# Autodesk Inventor assembly: Assem3omni
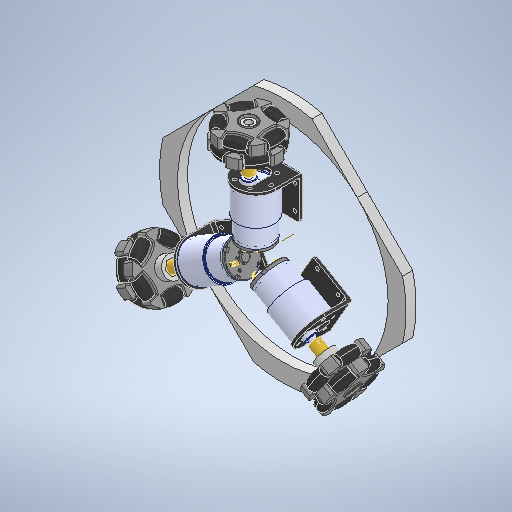
[picture p0: Inventor's stored thumbnail of the model, 512x512]
Saved by Autodesk Inventor 2025.1 (Build 291241000, 241)
## iProperties
Created: 2025-05-09
Part Number: Assem3omni
Document SubType Name: Assembly
Designer: User
Author: User
## Documents named in this file (3)
- D:\One Drive\OneDrive - Politeknik Sultan Salahuddin Abdul Aziz Shah\Documents\Inventor\RobosotPSA\Assem3omni.iam
- D:\One Drive\OneDrive - Politeknik Sultan Salahuddin Abdul Aziz Shah\Documents\Inventor\RobosotPSA\WheelMotor.iam
- D:\One Drive\OneDrive - Politeknik Sultan Salahuddin Abdul Aziz Shah\Documents\Inventor\RobosotPSA\MainBaseCircle210.ipt
## Components (4 placed, 2 different names)
1. MainBaseCircle210:1 — Flush:1
2. WheelMotor:1 [sub-assembly] — Flush:1
3. WheelMotor:2 [sub-assembly]
4. WheelMotor:3 [sub-assembly]
## Component patterns: (3 elements, first: WheelMotor:1)
## Relationships (1: Flush 1)
- Flush:1: MainBaseCircle210:1 ↔ WheelMotor:1
